# Autodesk Inventor assembly: 13361-30xxAE-08
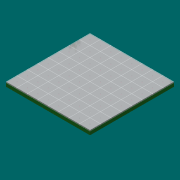
[picture p0: Inventor's stored thumbnail of the model, 180x180]
Saved by Autodesk Inventor 2016 (Build 200138000, 138)
## iProperties
Created: 2016-06-07
Part Number: 13361-30xxAE-08
Document SubType Name: Assembly
Designer: sawaiz
Author: sawaiz
## Documents named in this file (3)
- C:\Users\sawaiz\oneDrive\projects\modularRICH\dependency\13361-30xxAE-08\13361-30xxAE-08.iam
- C:\Users\sawaiz\oneDrive\projects\modularRICH\dependency\13361-30xxAE-08\13360-30xx-VE\13360-30xxVE.ipt
- C:\Users\sawaiz\oneDrive\projects\modularRICH\dependency\13361-30xxAE-08\backerBoardConnector.iam
## Components (65 placed, 2 different names)
1. backerBoardConnector:1 [sub-assembly] — Mate:1, Flush:1, Flush:2
2. 13360-30xxVE:1
3. 13360-30xxVE:2
4. 13360-30xxVE:3
5. 13360-30xxVE:4
6. 13360-30xxVE:5
7. 13360-30xxVE:6
8. 13360-30xxVE:7
9. 13360-30xxVE:8
10. 13360-30xxVE:9
11. 13360-30xxVE:10
12. 13360-30xxVE:11
13. 13360-30xxVE:12
14. 13360-30xxVE:13
15. 13360-30xxVE:14
16. 13360-30xxVE:15
17. 13360-30xxVE:16
18. 13360-30xxVE:17
19. 13360-30xxVE:18
20. 13360-30xxVE:19
21. 13360-30xxVE:20
22. 13360-30xxVE:21
23. 13360-30xxVE:22
24. 13360-30xxVE:23
25. 13360-30xxVE:24
26. 13360-30xxVE:25
27. 13360-30xxVE:26
28. 13360-30xxVE:27
29. 13360-30xxVE:28
30. 13360-30xxVE:29
31. 13360-30xxVE:30
32. 13360-30xxVE:31
33. 13360-30xxVE:32
34. 13360-30xxVE:33
35. 13360-30xxVE:34
36. 13360-30xxVE:35
37. 13360-30xxVE:36
38. 13360-30xxVE:37
39. 13360-30xxVE:38
40. 13360-30xxVE:39
41. 13360-30xxVE:40
42. 13360-30xxVE:41
43. 13360-30xxVE:42
44. 13360-30xxVE:43
45. 13360-30xxVE:44
46. 13360-30xxVE:45
47. 13360-30xxVE:46
48. 13360-30xxVE:47
49. 13360-30xxVE:48
50. 13360-30xxVE:49
51. 13360-30xxVE:50
52. 13360-30xxVE:51
53. 13360-30xxVE:52
54. 13360-30xxVE:53
55. 13360-30xxVE:54
56. 13360-30xxVE:55
57. 13360-30xxVE:56
58. 13360-30xxVE:57
59. 13360-30xxVE:58
60. 13360-30xxVE:59
61. 13360-30xxVE:60
62. 13360-30xxVE:61 — Mate:1
63. 13360-30xxVE:62
64. 13360-30xxVE:63 — Flush:1
65. 13360-30xxVE:64 — Flush:2
## Component patterns: (64 elements, first: 13360-30xxVE:1)
## Relationships (3: Flush 2, Mate 1)
- Mate:1: backerBoardConnector:1 ↔ 13360-30xxVE:61
- Flush:1: backerBoardConnector:1 ↔ 13360-30xxVE:63
- Flush:2: backerBoardConnector:1 ↔ 13360-30xxVE:64
